# Autodesk Inventor assembly: GA
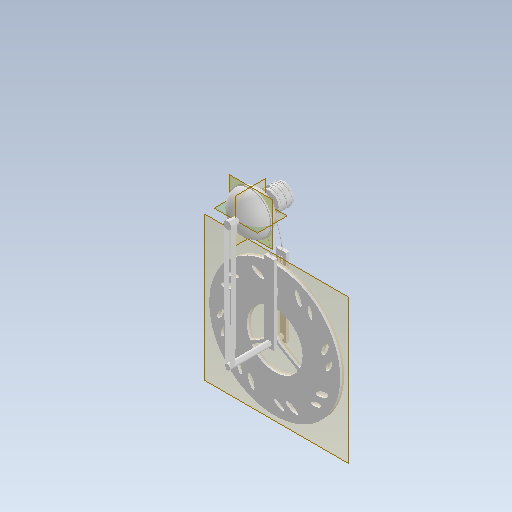
[picture p0: Inventor's stored thumbnail of the model, 512x512]
Saved by Autodesk Inventor 2020 (Build 240168000, 168)
## iProperties
Created: 2021-01-28
Part Number: GA
Document SubType Name: Assembly
Designer: kishore.balu
Project: LOCK
Description: General Assembly drawing
Engineer: LOKESH BABU/SRI SAI
Author: kishore.balu
Title: MABS-N
Revision Number: 0
## Documents named in this file (13)
- C:\Users\kishore.balu\Documents\LK\New folder\New folder\GA.iam
- C:\Users\kishore.balu\Documents\LK\New folder\disc.prt.ipt
- C:\Users\kishore.balu\Documents\LK\New folder\New folder\scissor.prt.ipt
- C:\Users\kishore.balu\Documents\LK\New folder\shoes.prt.ipt
- C:\Users\kishore.balu\Documents\LK\New folder\coupling_shaft.ipt
- C:\Users\kishore.balu\Documents\LK\New folder\coupling_sheel.ipt
- C:\Users\kishore.balu\Documents\LK\New folder\New folder\rod.ipt
- C:\Users\kishore.balu\Documents\LK\New folder\New folder\coupling_shaft3.ipt
- C:\Users\kishore.balu\Documents\LK\New folder\New folder\Thread.ipt
- C:\Users\kishore.balu\Documents\LK\New folder\New folder\Thread_MIR.ipt
- C:\Users\kishore.balu\Documents\LK\New folder\New folder\Belt.ipt
- C:\Users\kishore.balu\Documents\LK\New folder\New folder\Spring.ipt
- C:\Users\kishore.balu\Documents\LK\New folder\New folder\Spring_MIR.ipt
## Components (15 placed, 12 different names)
1. disc.prt:1 — Mate:1, Mate:2, Flush:1, Flush:2, Flush:4, Mate:14, Mate:17
2. scissor.prt:1 — Mate:1, Mate:2, Mate:4, Mate:3, Mate:5, Flush:3, Flush:5, Mate:22
3. shoes.prt:1 — Mate:4, Mate:3, Mate:5, Mate:30
4. coupling_shaft:1 — Flush:2, Flush:3, Flush:4, Mate:9, Mate:10, Mate:11, Mate:20, Mate:27
5. coupling_sheel:1 — Mate:9, Mate:10, Mate:12, Mate:27
6. coupling_sheel:2 — Mate:11, Mate:12, Mate:21
7. scissor.prt:2 — Mate:14, Mate:15, Mate:16, Mate:17, Mate:18, Mate:19, Mate:23
8. shoes.prt:2 — Mate:15, Mate:16, Mate:18, Mate:24
9. rod:1 — Mate:19, Flush:5, Mate:25
10. coupling_shaft3:1 — Mate:20, Mate:21, Mate:26, Mate:28
11. Thread:1 — Mate:22, Mate:23, Mate:24, Mate:29
12. Thread_MIR:1
13. Belt:1 — Mate:25, Mate:26, Mate:28
14. Spring:1 — Mate:29, Mate:30
15. Spring_MIR:1
## Relationships (31: Mate 26, Flush 5)
- Mate:1: disc.prt:1 ↔ scissor.prt:1
- Mate:2 (4 mm): disc.prt:1 ↔ scissor.prt:1
- Mate:4: scissor.prt:1 ↔ shoes.prt:1
- Mate:3: scissor.prt:1 ↔ shoes.prt:1
- Mate:5 (10 mm): scissor.prt:1 ↔ shoes.prt:1
- Flush:1 (-3 mm): disc.prt:1
- Flush:2 (-187.45 mm): disc.prt:1 ↔ coupling_shaft:1
- Flush:3: scissor.prt:1 ↔ coupling_shaft:1
- Flush:4: disc.prt:1 ↔ coupling_shaft:1
- Mate:9: coupling_shaft:1 ↔ coupling_sheel:1
- Mate:10 (-20.63 mm): coupling_shaft:1 ↔ coupling_sheel:1
- Mate:11: coupling_shaft:1 ↔ coupling_sheel:2
- Mate:12: coupling_sheel:1 ↔ coupling_sheel:2
- Mate:14 (4 mm): disc.prt:1 ↔ scissor.prt:2
- Mate:15: scissor.prt:2 ↔ shoes.prt:2
- Mate:16: scissor.prt:2 ↔ shoes.prt:2
- Mate:17: disc.prt:1 ↔ scissor.prt:2
- Mate:18 (10 mm): scissor.prt:2 ↔ shoes.prt:2
- Mate:19: scissor.prt:2 ↔ rod:1
- Flush:5: scissor.prt:1 ↔ rod:1
- Mate:20: coupling_shaft:1 ↔ coupling_shaft3:1
- Mate:21 (11.13 mm): coupling_sheel:2 ↔ coupling_shaft3:1
- Mate:22: scissor.prt:1 ↔ Thread:1
- Mate:23: scissor.prt:2 ↔ Thread:1
- Mate:24: shoes.prt:2 ↔ Thread:1
- Mate:25: rod:1 ↔ Belt:1
- Mate:26: coupling_shaft3:1 ↔ Belt:1
- Mate:27: coupling_shaft:1 ↔ coupling_sheel:1
- Mate:28: coupling_shaft3:1 ↔ Belt:1
- Mate:29: Thread:1 ↔ Spring:1
- Mate:30: shoes.prt:1 ↔ Spring:1
